# Autodesk Inventor assembly: primary-engineer-bench
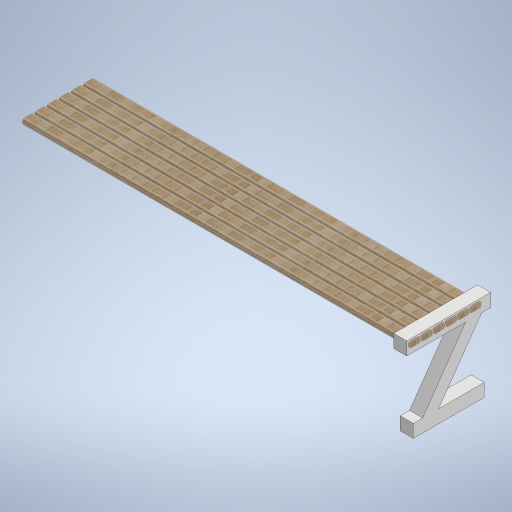
[picture p0: Inventor's stored thumbnail of the model, 512x512]
Saved by Autodesk Inventor 2023 (Build 270158030, 158C)
## iProperties
Created: 2024-09-09
Part Number: primary-engineer-bench
Document SubType Name: Assembly
Designer: Imogen Heard
Author: Imogen Heard
## Documents named in this file (3)
- C:\Users\dheard\Documents\0004-inventor\3D-CAD-main\primary-engineer-bench.iam
- C:\Users\dheard\Documents\0004-inventor\3D-CAD-main\bench-end-peice.ipt
- C:\Users\dheard\Documents\0004-inventor\3D-CAD-main\bench-slats.ipt
## Components (2 placed, 2 different names)
1. bench-end-peice:1 — Flush:1
2. bench-slats:1 — Flush:1
## Relationships (1: Flush 1)
- Flush:1: bench-end-peice:1 ↔ bench-slats:1
